# Autodesk Inventor assembly: Assembly1
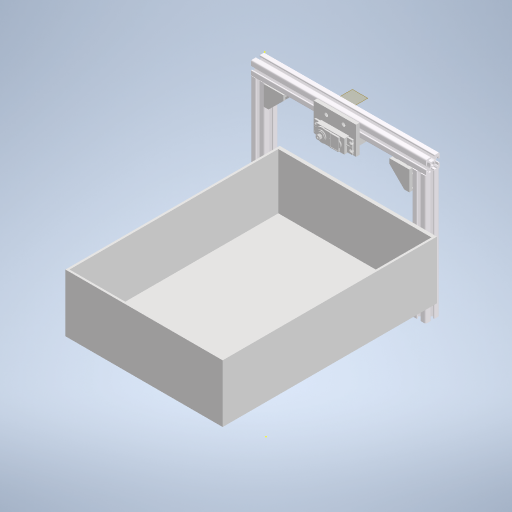
[picture p0: Inventor's stored thumbnail of the model, 512x512]
Saved by Autodesk Inventor 2023 (Build 270158000, 158)
## iProperties
Created: 2022-11-20
Part Number: Assembly1
Document SubType Name: Assembly
Designer: ADMIN
Author: ADMIN
## Documents named in this file (10)
- C:\Users\ADMIN\OneDrive\Máy tính\bản vẽ của Trung\Assembly1.iam
- C:\Users\ADMIN\OneDrive\Máy tính\bản vẽ của Trung\Nhom_dung.ipt
- C:\Users\ADMIN\OneDrive\Máy tính\bản vẽ của Trung\Nhom_ngang.ipt
- C:\Users\ADMIN\OneDrive\Máy tính\bản vẽ của Trung\MG 996R\MG996R.ipt
- C:\Users\ADMIN\OneDrive\Máy tính\bản vẽ của Trung\mieng_do_servo_5mm.ipt
- C:\Users\ADMIN\OneDrive\Máy tính\bản vẽ của Trung\al-20x20\corner_bracket_with_side_walls_20x20_rev2.ipt
- C:\Users\ADMIN\OneDrive\Máy tính\bản vẽ của Trung\mieng_mat_3mm.ipt
- C:\Users\ADMIN\OneDrive\Máy tính\bản vẽ của Trung\mieng_mat_5mm.ipt
- C:\Users\ADMIN\OneDrive\Máy tính\bản vẽ của Trung\totalPart.ipt
- C:\Users\ADMIN\OneDrive\Máy tính\bản vẽ của Trung\mieng_ben_3mm.ipt
## Components (12 placed, 9 different names)
1. Nhom_dung:1 — Mate:2, Tangent:3, Tangent:4, Mate:10
2. Nhom_dung:2 — Flush:1, Mate:1, Mate:8
3. Nhom_ngang:1 — Mate:1, Mate:2, Mate:3, Mate:9, Tangent:1, Tangent:2, Tangent:5, Tangent:6, Mate:11
4. MG996R:1 — Mate:4, Mate:5
5. mieng_do_servo_5mm:1 — Mate:3, Mate:4, Mate:5
6. corner_bracket_with_side_walls_20x20_rev2:1 — Mate:8, Mate:9, Tangent:1, Tangent:2
7. corner_bracket_with_side_walls_20x20_rev2:2 — Tangent:3, Tangent:4, Mate:10, Tangent:5, Tangent:6, Mate:11
8. totalPart:1 — Mate:12, Mate:13, Mate:14, Mate:15, Mate:16, Mate:17, Mate:18, Mate:19, Mate:20, Mate:21, Mate:22, Mate:23
9. mieng_ben_3mm:1 — Mate:12, Mate:13, Mate:14
10. mieng_ben_3mm:2 — Mate:15, Mate:16, Mate:17
11. mieng_mat_3mm:2 — Mate:18, Mate:19, Mate:20
12. mieng_mat_5mm:1 — Mate:21, Mate:22, Mate:23
## Relationships (28: Mate 21, Tangent 6, Flush 1)
- Flush:1: Nhom_dung:2
- Mate:1: Nhom_dung:2 ↔ Nhom_ngang:1
- Mate:2: Nhom_dung:1 ↔ Nhom_ngang:1
- Mate:3: Nhom_ngang:1 ↔ mieng_do_servo_5mm:1
- Mate:4: MG996R:1 ↔ mieng_do_servo_5mm:1
- Mate:5: MG996R:1 ↔ mieng_do_servo_5mm:1
- Mate:8: Nhom_dung:2 ↔ corner_bracket_with_side_walls_20x20_rev2:1
- Mate:9: Nhom_ngang:1 ↔ corner_bracket_with_side_walls_20x20_rev2:1
- Tangent:1: Nhom_ngang:1 ↔ corner_bracket_with_side_walls_20x20_rev2:1
- Tangent:2: Nhom_ngang:1 ↔ corner_bracket_with_side_walls_20x20_rev2:1
- Tangent:3: Nhom_dung:1 ↔ corner_bracket_with_side_walls_20x20_rev2:2
- Tangent:4: Nhom_dung:1 ↔ corner_bracket_with_side_walls_20x20_rev2:2
- Mate:10: Nhom_dung:1 ↔ corner_bracket_with_side_walls_20x20_rev2:2
- Tangent:5: Nhom_ngang:1 ↔ corner_bracket_with_side_walls_20x20_rev2:2
- Tangent:6: Nhom_ngang:1 ↔ corner_bracket_with_side_walls_20x20_rev2:2
- Mate:11: Nhom_ngang:1 ↔ corner_bracket_with_side_walls_20x20_rev2:2
- Mate:12: totalPart:1 ↔ mieng_ben_3mm:1
- Mate:13: totalPart:1 ↔ mieng_ben_3mm:1
- Mate:14: totalPart:1 ↔ mieng_ben_3mm:1
- Mate:15: totalPart:1 ↔ mieng_ben_3mm:2
- Mate:16: totalPart:1 ↔ mieng_ben_3mm:2
- Mate:17: totalPart:1 ↔ mieng_ben_3mm:2
- Mate:18: totalPart:1 ↔ mieng_mat_3mm:2
- Mate:19: totalPart:1 ↔ mieng_mat_3mm:2
- Mate:20: totalPart:1 ↔ mieng_mat_3mm:2
- Mate:21: totalPart:1 ↔ mieng_mat_5mm:1
- Mate:22: totalPart:1 ↔ mieng_mat_5mm:1
- Mate:23: totalPart:1 ↔ mieng_mat_5mm:1
